# Autodesk Inventor assembly: A1 test 1
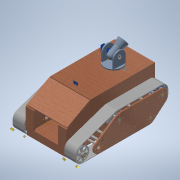
[picture p0: Inventor's stored thumbnail of the model, 180x180]
Saved by Autodesk Inventor 2021 (Build 250183000, 183)
## iProperties
Manager: PJ / DCS
Company: Emmaüs Bovenbouw Aalter
Created: 2021-01-09
Part Number: A1 test 1
Catalog Web Link: http://emmausbovenbouw.op-weg.be/
Vendor: Emmaüs Bovenbouw Aalter
Document SubType Name: Assembly
Designer: Antho
Engineer: Declercq St.
Authority: Declercq St.
Title: Algemene Projecttitel
Author: Antho
## Documents named in this file (15)
- C:\Users\Antho\OneDrive\Documenten\Inventor\Inventor\GIP 6EM\Assembly\A1\A1 test 1.iam
- C:\Users\Antho\OneDrive\Documenten\Inventor\Inventor\GIP 6EM\Frame\Plaat achter.ipt
- C:\Users\Antho\OneDrive\Documenten\Inventor\Inventor\GIP 6EM\Wielen\Frame wiel binnen.ipt
- C:\Users\Antho\OneDrive\Documenten\Inventor\Inventor\GIP 6EM\Bevestigingen\Ball Bearing\W 619_6-2Z.iam
- C:\Users\Antho\OneDrive\Documenten\Inventor\Inventor\GIP 6EM\steunstuk\Steun stuk.ipt
- C:\Users\Antho\OneDrive\Documenten\Inventor\Inventor\GIP 6EM\Assembly\Assembly tandwiel.iam
- C:\Users\Antho\OneDrive\Documenten\Inventor\Inventor\GIP 6EM\Assembly\Assembly wiel.iam
- C:\Users\Antho\OneDrive\Documenten\Inventor\Inventor\GIP 6EM\Wielen\Rupsband.ipt
- C:\Users\Antho\OneDrive\Documenten\Inventor\Inventor\GIP 6EM\Wielen\Frame wiel.ipt
- C:\Users\Antho\OneDrive\Documenten\Inventor\Inventor\GIP 6EM\Wielen\DC motor connectie.ipt
- C:\Users\Antho\OneDrive\Documenten\Inventor\Inventor\GIP 6EM\Wielen\DC motor connectie part 2.ipt
- C:\Users\Antho\OneDrive\Documenten\Inventor\Inventor\GIP 6EM\waterkannon\Samenstel waterkanon januari.iam
- C:\Users\Antho\OneDrive\Documenten\Inventor\Inventor\GIP 6EM\Frame\schuine plaat.ipt
- C:\Users\Antho\OneDrive\Documenten\Inventor\Inventor\GIP 6EM\Assembly\Assembly esp32.iam
- C:\Users\Antho\OneDrive\Documenten\Inventor\Inventor\GIP 6EM\Assembly\assambly onderplaat A.iam
## Components (51 placed, 14 different names)
1. Plaat achter:1 — Flush:3, Mate:92, Flush:34, Flush:35, Flush:36, Mate:94, Flush:37, Mate:96
2. Frame wiel binnen:1 — Mate:49, Mate:50, Mate:51, Mate:52, Flush:22, Flush:23, Flush:24, Flush:25, Mate:53, Mate:54, Mate:55, Mate:56, Mate:57, Mate:58, Mate:59, Mate:60, Mate:61, Mate:62, Mate:63, Mate:64, Mate:65, Mate:66, Mate:72, Mate:73, Mate:74, Mate:81, Mate:85, Mate:92, Flush:34, Flush:35, Flush:40
3. Frame wiel binnen:2 — Flush:3, Mate:9, Mate:10, Mate:11, Mate:12, Flush:8, Flush:9, Flush:10, Flush:11, Mate:13, Mate:14, Mate:15, Mate:16, Mate:17, Mate:18, Mate:19, Mate:20, Mate:21, Mate:22, Mate:23, Mate:24, Mate:25, Mate:26, Flush:12, Flush:14, Flush:15, Mate:32, Mate:43, Flush:20, Mate:86, Mate:87, Flush:30, Mate:90, Flush:31, Flush:32, Mate:91, Flush:37, Mate:95, Flush:41, Mate:96
4. W 619_6-2Z:1 [sub-assembly] — Mate:9, Flush:11, Mate:31
5. W 619_6-2Z:2 [sub-assembly] — Mate:10, Flush:10, Mate:28
6. W 619_6-2Z:3 [sub-assembly] — Mate:11, Flush:9, Mate:30
7. W 619_6-2Z:4 [sub-assembly] — Mate:12, Flush:8, Mate:29
8. Steun stuk:1 — Mate:15, Mate:21
9. Steun stuk:2 — Mate:16, Mate:25
10. Steun stuk:3 — Mate:14, Mate:20
11. Steun stuk:4 — Mate:19, Mate:22
12. Steun stuk:5 — Mate:18, Mate:24
13. Steun stuk:6 — Mate:17, Mate:23
14. Steun stuk:7 — Mate:13, Mate:26, Mate:36
15. Assembly tandwiel:1 [sub-assembly] — Mate:30, Mate:40, Flush:16, Flush:20
16. Assembly wiel:1 [sub-assembly] — Mate:28, Flush:14, Mate:35, Mate:38, Flush:18
17. Assembly wiel:2 [sub-assembly] — Mate:29, Flush:12, Mate:39, Flush:17
18. Assembly wiel:3 [sub-assembly] — Mate:31, Flush:15, Mate:34, Mate:37, Flush:19
19. Rupsband:1 — Mate:32, Mate:34, Mate:35
20. Frame wiel:1 — Mate:36, Mate:41, Mate:42
21. W 619_6-2Z:5 [sub-assembly] — Mate:40, Flush:16, Mate:42
22. W 619_6-2Z:6 [sub-assembly] — Mate:39, Flush:17
23. W 619_6-2Z:7 [sub-assembly] — Mate:38, Flush:18
24. W 619_6-2Z:8 [sub-assembly] — Mate:37, Flush:19, Mate:41
25. DC motor connectie:1 — Mate:43, Mate:44
26. DC motor connectie part 2:1 — Mate:44
27. Samenstel waterkanon januari:1 [sub-assembly] — Mate:88, Mate:89, Flush:30, Mate:90, Flush:31, Flush:39, Flush:40, Mate:95, Flush:41, Flush:42
28. W 619_6-2Z:9 [sub-assembly] — Mate:52, Flush:24, Mate:67, Mate:68
29. W 619_6-2Z:10 [sub-assembly] — Mate:50, Flush:25, Mate:71
30. W 619_6-2Z:11 [sub-assembly] — Mate:49, Flush:22, Mate:70
31. W 619_6-2Z:12 [sub-assembly] — Mate:51, Flush:23, Mate:69
32. Steun stuk:8 — Mate:59, Mate:61
33. Steun stuk:9 — Mate:54, Mate:66
34. Steun stuk:10 — Mate:55, Mate:64, Mate:84
35. Steun stuk:11 — Mate:57, Mate:60
36. Steun stuk:12 — Mate:53, Mate:65
37. Steun stuk:13 — Mate:58, Mate:62
38. Steun stuk:14 — Mate:56, Mate:63
39. Assembly tandwiel:2 [sub-assembly] — Mate:67, Mate:68, Mate:78, Flush:27
40. Assembly wiel:4 [sub-assembly] — Mate:69, Mate:72, Mate:77, Flush:28, Mate:80
41. Assembly wiel:5 [sub-assembly] — Mate:70, Mate:73, Mate:76, Flush:29
42. Assembly wiel:6 [sub-assembly] — Mate:71, Mate:74, Mate:75, Flush:26, Mate:79
43. W 619_6-2Z:13 [sub-assembly] — Mate:78, Flush:27, Mate:82
44. W 619_6-2Z:14 [sub-assembly] — Mate:75, Flush:26, Mate:83
45. W 619_6-2Z:15 [sub-assembly] — Mate:76, Flush:29
46. W 619_6-2Z:16 [sub-assembly] — Mate:77, Flush:28
47. Rupsband:2 — Mate:79, Mate:80, Mate:81
48. Frame wiel:2 — Mate:82, Mate:83, Mate:84
49. schuine plaat:1 — Mate:85, Mate:86, Mate:87
50. Assembly esp32:1 [sub-assembly] — Mate:88, Mate:89, Flush:32, Flush:39, Flush:42
51. assambly onderplaat A:1 [sub-assembly] — Mate:91, Flush:36, Mate:94
## Relationships (113: Mate 81, Flush 32)
- Flush:3: Plaat achter:1 ↔ Frame wiel binnen:2
- Mate:9: Frame wiel binnen:2 ↔ W 619_6-2Z:1
- Mate:10: Frame wiel binnen:2 ↔ W 619_6-2Z:2
- Mate:11: Frame wiel binnen:2 ↔ W 619_6-2Z:3
- Mate:12: Frame wiel binnen:2 ↔ W 619_6-2Z:4
- Flush:8: Frame wiel binnen:2 ↔ W 619_6-2Z:4
- Flush:9: Frame wiel binnen:2 ↔ W 619_6-2Z:3
- Flush:10: Frame wiel binnen:2 ↔ W 619_6-2Z:2
- Flush:11: Frame wiel binnen:2 ↔ W 619_6-2Z:1
- Mate:13: Frame wiel binnen:2 ↔ Steun stuk:7
- Mate:14: Frame wiel binnen:2 ↔ Steun stuk:3
- Mate:15: Frame wiel binnen:2 ↔ Steun stuk:1
- Mate:16: Frame wiel binnen:2 ↔ Steun stuk:2
- Mate:17: Frame wiel binnen:2 ↔ Steun stuk:6
- Mate:18: Frame wiel binnen:2 ↔ Steun stuk:5
- Mate:19: Frame wiel binnen:2 ↔ Steun stuk:4
- Mate:20: Frame wiel binnen:2 ↔ Steun stuk:3
- Mate:21: Frame wiel binnen:2 ↔ Steun stuk:1
- Mate:22: Frame wiel binnen:2 ↔ Steun stuk:4
- Mate:23: Frame wiel binnen:2 ↔ Steun stuk:6
- Mate:24: Frame wiel binnen:2 ↔ Steun stuk:5
- Mate:25: Frame wiel binnen:2 ↔ Steun stuk:2
- Mate:26: Frame wiel binnen:2 ↔ Steun stuk:7
- Mate:28: W 619_6-2Z:2 ↔ Assembly wiel:1
- Mate:29: W 619_6-2Z:4 ↔ Assembly wiel:2
- Mate:30: W 619_6-2Z:3 ↔ Assembly tandwiel:1
- Mate:31: W 619_6-2Z:1 ↔ Assembly wiel:3
- Flush:12: Frame wiel binnen:2 ↔ Assembly wiel:2
- Flush:14: Frame wiel binnen:2 ↔ Assembly wiel:1
- Flush:15: Frame wiel binnen:2 ↔ Assembly wiel:3
- Mate:32: Frame wiel binnen:2 ↔ Rupsband:1
- Mate:34: Assembly wiel:3 ↔ Rupsband:1
- Mate:35: Assembly wiel:1 ↔ Rupsband:1
- Mate:36: Steun stuk:7 ↔ Frame wiel:1
- Mate:37: Assembly wiel:3 ↔ W 619_6-2Z:8
- Mate:38: Assembly wiel:1 ↔ W 619_6-2Z:7
- Mate:39: Assembly wiel:2 ↔ W 619_6-2Z:6
- Mate:40: Assembly tandwiel:1 ↔ W 619_6-2Z:5
- Flush:16: Assembly tandwiel:1 ↔ W 619_6-2Z:5
- Flush:17: Assembly wiel:2 ↔ W 619_6-2Z:6
- Flush:18: Assembly wiel:1 ↔ W 619_6-2Z:7
- Flush:19: Assembly wiel:3 ↔ W 619_6-2Z:8
- Mate:41: Frame wiel:1 ↔ W 619_6-2Z:8
- Mate:42: Frame wiel:1 ↔ W 619_6-2Z:5
- Mate:43: Frame wiel binnen:2 ↔ DC motor connectie:1
- Flush:20: Frame wiel binnen:2 ↔ Assembly tandwiel:1
- Mate:44: DC motor connectie:1 ↔ DC motor connectie part 2:1
- Mate:49: Frame wiel binnen:1 ↔ W 619_6-2Z:11
- Mate:50: Frame wiel binnen:1 ↔ W 619_6-2Z:10
- Mate:51: Frame wiel binnen:1 ↔ W 619_6-2Z:12
- Mate:52: Frame wiel binnen:1 ↔ W 619_6-2Z:9
- Flush:22: Frame wiel binnen:1 ↔ W 619_6-2Z:11
- Flush:23: Frame wiel binnen:1 ↔ W 619_6-2Z:12
- Flush:24: Frame wiel binnen:1 ↔ W 619_6-2Z:9
- Flush:25: Frame wiel binnen:1 ↔ W 619_6-2Z:10
- Mate:53: Frame wiel binnen:1 ↔ Steun stuk:12
- Mate:54: Frame wiel binnen:1 ↔ Steun stuk:9
- Mate:55: Frame wiel binnen:1 ↔ Steun stuk:10
- Mate:56: Frame wiel binnen:1 ↔ Steun stuk:14
- Mate:57: Frame wiel binnen:1 ↔ Steun stuk:11
- Mate:58: Frame wiel binnen:1 ↔ Steun stuk:13
- Mate:59: Frame wiel binnen:1 ↔ Steun stuk:8
- Mate:60: Frame wiel binnen:1 ↔ Steun stuk:11
- Mate:61: Frame wiel binnen:1 ↔ Steun stuk:8
- Mate:62: Frame wiel binnen:1 ↔ Steun stuk:13
- Mate:63: Frame wiel binnen:1 ↔ Steun stuk:14
- Mate:64: Frame wiel binnen:1 ↔ Steun stuk:10
- Mate:65: Frame wiel binnen:1 ↔ Steun stuk:12
- Mate:66: Frame wiel binnen:1 ↔ Steun stuk:9
- Mate:67: W 619_6-2Z:9 ↔ Assembly tandwiel:2
- Mate:68: W 619_6-2Z:9 ↔ Assembly tandwiel:2
- Mate:69: W 619_6-2Z:12 ↔ Assembly wiel:4
- Mate:70: W 619_6-2Z:11 ↔ Assembly wiel:5
- Mate:71: W 619_6-2Z:10 ↔ Assembly wiel:6
- Mate:72: Frame wiel binnen:1 ↔ Assembly wiel:4
- Mate:73: Frame wiel binnen:1 ↔ Assembly wiel:5
- Mate:74: Frame wiel binnen:1 ↔ Assembly wiel:6
- Mate:75: Assembly wiel:6 ↔ W 619_6-2Z:14
- Flush:26: Assembly wiel:6 ↔ W 619_6-2Z:14
- Mate:76: Assembly wiel:5 ↔ W 619_6-2Z:15
- Mate:77: Assembly wiel:4 ↔ W 619_6-2Z:16
- Mate:78: Assembly tandwiel:2 ↔ W 619_6-2Z:13
- Flush:27: Assembly tandwiel:2 ↔ W 619_6-2Z:13
- Flush:28: Assembly wiel:4 ↔ W 619_6-2Z:16
- Flush:29: Assembly wiel:5 ↔ W 619_6-2Z:15
- Mate:79: Assembly wiel:6 ↔ Rupsband:2
- Mate:80: Assembly wiel:4 ↔ Rupsband:2
- Mate:81: Frame wiel binnen:1 ↔ Rupsband:2
- Mate:82: W 619_6-2Z:13 ↔ Frame wiel:2
- Mate:83: W 619_6-2Z:14 ↔ Frame wiel:2
- Mate:84: Steun stuk:10 ↔ Frame wiel:2
- Mate:85: Frame wiel binnen:1 ↔ schuine plaat:1
- Mate:86: Frame wiel binnen:2 ↔ schuine plaat:1
- Mate:87 (0.25 mm): Frame wiel binnen:2 ↔ schuine plaat:1
- Mate:88: Samenstel waterkanon januari:1 ↔ Assembly esp32:1
- Mate:89: Samenstel waterkanon januari:1 ↔ Assembly esp32:1
- Flush:30: Frame wiel binnen:2 ↔ Samenstel waterkanon januari:1
- Mate:90: Frame wiel binnen:2 ↔ Samenstel waterkanon januari:1
- Flush:31: Frame wiel binnen:2 ↔ Samenstel waterkanon januari:1
- Flush:32: Frame wiel binnen:2 ↔ Assembly esp32:1
- Mate:91: Frame wiel binnen:2 ↔ assambly onderplaat A:1
- Mate:92: Plaat achter:1 ↔ Frame wiel binnen:1
- Flush:34: Plaat achter:1 ↔ Frame wiel binnen:1
- Flush:35: Plaat achter:1 ↔ Frame wiel binnen:1
- Flush:36: Plaat achter:1 ↔ assambly onderplaat A:1
- Mate:94: Plaat achter:1 ↔ assambly onderplaat A:1
- Flush:37: Plaat achter:1 ↔ Frame wiel binnen:2
- Flush:39: Samenstel waterkanon januari:1 ↔ Assembly esp32:1
- Flush:40: Frame wiel binnen:1 ↔ Samenstel waterkanon januari:1
- Mate:95: Frame wiel binnen:2 ↔ Samenstel waterkanon januari:1
- Flush:41: Frame wiel binnen:2 ↔ Samenstel waterkanon januari:1
- Flush:42: Samenstel waterkanon januari:1 ↔ Assembly esp32:1
- Mate:96: Plaat achter:1 ↔ Frame wiel binnen:2
